# Autodesk Inventor assembly: CoaxialSPM
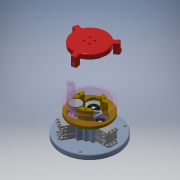
[picture p0: Inventor's stored thumbnail of the model, 180x180]
Saved by Autodesk Inventor 2019 (Build 230136000, 136)
## iProperties
Created: 2022-08-24
Part Number: CoaxialSPM
Document SubType Name: Assembly
Designer: zreik
Author: zreik
## Documents named in this file (9)
- D:\Documents\HIAST\4th year\4th Year Project\Design\Coaxial\CoaxialSPM.iam
- D:\Documents\HIAST\4th year\4th Year Project\Design\Coaxial\Base.ipt
- D:\Documents\HIAST\4th year\4th Year Project\Design\Coaxial\LayerBase.ipt
- D:\Documents\HIAST\4th year\4th Year Project\Design\Coaxial\Layer2Gear.ipt
- D:\Documents\HIAST\4th year\4th Year Project\Design\Coaxial\Layer3Gear.ipt
- D:\Documents\HIAST\4th year\4th Year Project\Design\Coaxial\LayerGear.ipt
- D:\Documents\HIAST\4th year\4th Year Project\Design\Coaxial\TopPlatform.ipt
- D:\Documents\HIAST\4th year\4th Year Project\Design\Coaxial\XL-320.ipt
- D:\Documents\HIAST\4th year\4th Year Project\Design\Coaxial\Motor1Gear.ipt
## Components (12 placed, 8 different names)
1. Base:1 — Mate:1, Flush:1, Mate:2, Mate:7, Mate:11, Mate:29, Mate:33, Mate:34, Mate:35, Mate:36, Mate:37, Mate:38, Mate:39, Mate:40, Mate:41
2. LayerBase:1 — Mate:3, Mate:4, Mate:6, Mate:9, Mate:11, Mate:16, Mate:17
3. LayerBase:2 — Mate:3, Mate:5, Mate:7, Mate:8, Mate:12, Mate:13, Mate:29
4. LayerBase:3 — Mate:4, Mate:5, Mate:6, Mate:8, Mate:9, Mate:14, Mate:15
5. Layer1Gear:1 — Mate:12, Mate:13, Mate:19
6. Layer2Gear:1 — Mate:14, Mate:15, Mate:18
7. Layer3Gear:1 — Mate:16, Mate:17, Mate:20, Angle:1
8. TopPlatform:1 — Mate:23, Mate:24, Mate:25, Angle:1
9. XL-320:1 — Mate:39, Mate:40, Mate:41
10. XL-320:2 — Mate:36, Mate:37, Mate:38
11. XL-320:3 — Mate:30, Mate:31, Mate:32, Mate:33, Mate:34, Mate:35
12. Motor1Gear:1 — Mate:30, Mate:31, Mate:32
## Relationships (42: Mate 40, Flush 1, Angle 1)
- Mate:1: Base:1
- Flush:1: Base:1
- Mate:2: Base:1
- Mate:3: LayerBase:1 ↔ LayerBase:2
- Mate:4: LayerBase:1 ↔ LayerBase:3
- Mate:5: LayerBase:2 ↔ LayerBase:3
- Mate:6: LayerBase:1 ↔ LayerBase:3
- Mate:7: Base:1 ↔ LayerBase:2
- Mate:8: LayerBase:2 ↔ LayerBase:3
- Mate:9: LayerBase:1 ↔ LayerBase:3
- Mate:11: Base:1 ↔ LayerBase:1
- Mate:12: LayerBase:2 ↔ Layer1Gear:1
- Mate:13: LayerBase:2 ↔ Layer1Gear:1
- Mate:14: LayerBase:3 ↔ Layer2Gear:1
- Mate:15: LayerBase:3 ↔ Layer2Gear:1
- Mate:16: LayerBase:1 ↔ Layer3Gear:1
- Mate:17: LayerBase:1 ↔ Layer3Gear:1
- Mate:18: Layer2Gear:1
- Mate:19: Layer1Gear:1
- Mate:20: Layer3Gear:1
- Mate:21
- Mate:22
- Mate:23: TopPlatform:1
- Mate:24: TopPlatform:1
- Mate:25: TopPlatform:1
- Mate:26
- Mate:27
- Mate:28
- Angle:1 (0 deg): Layer3Gear:1 ↔ TopPlatform:1
- Mate:29: Base:1 ↔ LayerBase:2
- Mate:30: XL-320:3 ↔ Motor1Gear:1
- Mate:31: XL-320:3 ↔ Motor1Gear:1
- Mate:32: XL-320:3 ↔ Motor1Gear:1
- Mate:33: Base:1 ↔ XL-320:3
- Mate:34: Base:1 ↔ XL-320:3
- Mate:35: Base:1 ↔ XL-320:3
- Mate:36: Base:1 ↔ XL-320:2
- Mate:37: Base:1 ↔ XL-320:2
- Mate:38: Base:1 ↔ XL-320:2
- Mate:39: Base:1 ↔ XL-320:1
- Mate:40: Base:1 ↔ XL-320:1
- Mate:41: Base:1 ↔ XL-320:1
